# Autodesk Inventor assembly: Screw_Joint_36T_MIR2
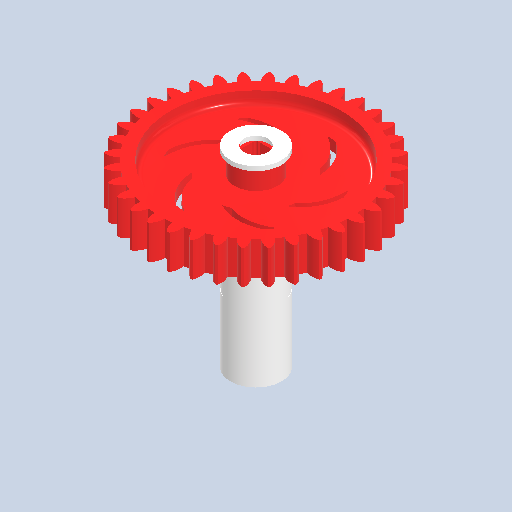
[picture p0: Inventor's stored thumbnail of the model, 512x512]
Saved by Autodesk Inventor 2025.2 (Build 292293000, 293)
## iProperties
Created: 2024-12-08
Part Number: Screw_Joint_36T_MIR2
Document SubType Name: Assembly
Designer: joshi
Author: Aditya Koduri
## Documents named in this file (6)
- C:\Users\joshi\Desktop\3388K CAD\Screw_Joint_36T_MIR2.iam
- C:\Users\joshi\Desktop\3388K CAD\VEX Main\Motion\Gears\LS 36T Gear_MIR2.ipt
- C:\Users\joshi\Desktop\3388K CAD\VEX Main\Motion\Spacers\Washer Teflon\TWasher .375 OD x .03125.ipt
- C:\Users\joshi\Desktop\3388K CAD\VEX Main\Motion\Spacers\Washer Teflon.ipt
- C:\Users\joshi\Desktop\3388K CAD\VEX Main\Motion\Spacers\Spacer Nylon .313 OD\NSpacer .313 OD x .500.ipt
- C:\Users\joshi\Desktop\3388K CAD\VEX Main\Motion\Spacers\Spacer Nylon .313 OD.ipt
## Components (4 placed, 3 different names)
1. LS 36T Gear_MIR2:1 — Insert:1, Insert:2
2. TWasher .375 OD x .03125:1 — Insert:1
3. NSpacer .313 OD x .500:1 — Insert:2, Insert:3
4. NSpacer .313 OD x .500:2 — Insert:3
## Relationships (3: Insert 3)
- Insert:1: LS 36T Gear_MIR2:1 ↔ TWasher .375 OD x .03125:1
- Insert:2: LS 36T Gear_MIR2:1 ↔ NSpacer .313 OD x .500:1
- Insert:3: NSpacer .313 OD x .500:1 ↔ NSpacer .313 OD x .500:2
